# Autodesk Inventor assembly: 0005-00-02 X axis
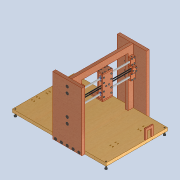
[picture p0: Inventor's stored thumbnail of the model, 180x180]
Saved by Autodesk Inventor 2020 (Build 240168000, 168)
## iProperties
Created: 2020-12-18
Part Number: 0005-00-02 X axis
Document SubType Name: Assembly
Designer: Iulian Bors
Mass: 17144.8 g
Surface Area: 27601.7 cm^2
Volume: 16303.9 cm^3
Density: 1.05157 g/cm^3
Author: Iulian Bors
## Documents named in this file (22)
- Z:\I.A.B\Proiecte\0005 I.A.B 3d 2.0 Imprimanta aracet\10 Mecanic\0005-00-02 X axis.iam
- Z:\I.A.B\Proiecte\0005 I.A.B 3d 2.0 Imprimanta aracet\10 Mecanic\0005-10-011.ipt
- Z:\I.A.B\Proiecte\0005 I.A.B 3d 2.0 Imprimanta aracet\10 Mecanic\0005-10-012.ipt
- Z:\I.A.B\Proiecte\0005 I.A.B 3d 2.0 Imprimanta aracet\10 Mecanic\0005-10-1009 LM10uu.ipt
- Z:\I.A.B\Proiecte\0005 I.A.B 3d 2.0 Imprimanta aracet\10 Mecanic\Surub M4 saiba piulita.iam
- Z:\I.A.B\Proiecte\0005 I.A.B 3d 2.0 Imprimanta aracet\10 Mecanic\0005-10-027 suport nema Z.ipt
- Z:\I.A.B\Proiecte\0005 I.A.B 3d 2.0 Imprimanta aracet\10 Mecanic\0005-10-1007 Bara rectificata.ipt
- Z:\I.A.B\Proiecte\0005 I.A.B 3d 2.0 Imprimanta aracet\10 Mecanic\0005-10-015 suport tija.ipt
- Z:\I.A.B\Proiecte\0005 I.A.B 3d 2.0 Imprimanta aracet\10 Mecanic\0005-10-1001 NEMA17 - Motor de passo.ipt
- Z:\I.A.B\Proiecte\0005 I.A.B 3d 2.0 Imprimanta aracet\10 Mecanic\0005-10-1010 GT2 Timing Pulley 20 Tooth.ipt
- Z:\I.A.B\Proiecte\0005 I.A.B 3d 2.0 Imprimanta aracet\10 Mecanic\0005-10-1011 16T W6 B3 Without T_Shrinkwrap_1.ipt
- Z:\I.A.B\Proiecte\0005 I.A.B 3d 2.0 Imprimanta aracet\10 Mecanic\0005-10-018 intinzator x.ipt
- Z:\I.A.B\Proiecte\0005 I.A.B 3d 2.0 Imprimanta aracet\10 Mecanic\0005-10-1015 curea x.ipt
- Z:\I.A.B\Proiecte\0005 I.A.B 3d 2.0 Imprimanta aracet\10 Mecanic\0005-10-023 Suport motor x.ipt
- C:\Users\40743\Documents\Inventor\Content Center Files\R2020\en-US\ISO 7050 - C-Z(2)\ISO 7050 - ST 3.5 x 22 - C - Z.ipt
- Z:\I.A.B\Proiecte\0005 I.A.B 3d 2.0 Imprimanta aracet\10 Mecanic\0005-10-01 Cadru.iam
- Z:\I.A.B\Proiecte\0005 I.A.B 3d 2.0 Imprimanta aracet\10 Mecanic\Surub M4 saiba piulita 50mm.iam
- Z:\I.A.B\Proiecte\0005 I.A.B 3d 2.0 Imprimanta aracet\10 Mecanic\0005-10-1030 DIN 933 - M4  x 20.ipt
- Z:\I.A.B\Proiecte\0005 I.A.B 3d 2.0 Imprimanta aracet\10 Mecanic\Surub M4 saiba piulita 60mm.iam
- Z:\I.A.B\Proiecte\0005 I.A.B 3d 2.0 Imprimanta aracet\10 Mecanic\0005-10-1032.ipt
- Z:\I.A.B\Proiecte\0005 I.A.B 3d 2.0 Imprimanta aracet\10 Mecanic\0005-10-1020 ISO 7089 - 3 - 140 HV(1).ipt
- Z:\I.A.B\Proiecte\0005 I.A.B 3d 2.0 Imprimanta aracet\10 Mecanic\0005-10-1033 DIN 914 - M5 x 10.ipt
## Components (82 placed, 21 different names)
1. 0005-10-011.ipt:20 — Flush:69, Flush:70, Mate:151, Insert:33, Insert:34
2. 0005-10-011.ipt:24 — Mate:142, Flush:71, Flush:72, Insert:35, Insert:36
3. 0005-10-012.ipt:25 — Flush:22, Flush:25, Flush:26, Mate:40, Mate:56, Mate:57, Mate:71, Mate:72, Flush:44, Mate:142, Mate:151
4. 0005-10-1009 LM10uu.ipt:28 — Flush:22, Mate:49, Mate:56, Mate:57
5. 0005-10-012.ipt:29 — Flush:25, Flush:34, Flush:26, Mate:40, Insert:18, Insert:19, Flush:69, Flush:70, Flush:71, Flush:72, Insert:21, Insert:22, Insert:24, Insert:25, Insert:27, Insert:28, Insert:30, Insert:40
6. 0005-10-1009 LM10uu.ipt:37 — Mate:49, Flush:34, Flush:45, Mate:172
7. 0005-10-1009 LM10uu.ipt:53 — Mate:71, Mate:72, Flush:44, Mate:73
8. 0005-10-1009 LM10uu.ipt:54 — Flush:45, Mate:73, Mate:164
9. Surub M4 saiba piulita.iam:65 [sub-assembly] — Insert:18
10. Surub M4 saiba piulita.iam:67 [sub-assembly] — Insert:19
11. Surub M4 saiba piulita:7 [sub-assembly] — Insert:21
12. Surub M4 saiba piulita:8 [sub-assembly] — Insert:22
13. Surub M4 saiba piulita:10 [sub-assembly] — Insert:24
14. Surub M4 saiba piulita:11 [sub-assembly] — Insert:27
15. Surub M4 saiba piulita:12 [sub-assembly] — Insert:25
16. Surub M4 saiba piulita:15 [sub-assembly] — Insert:28
17. Surub M4 saiba piulita:17 [sub-assembly] — Insert:30
18. 0005-10-1007 Bara rectificata:1 — Mate:172, Mate:173, Flush:75, Mate:176, Flush:77
19. 0005-10-015 suport tija:1 — Mate:165, Mate:166, Mate:167, Mate:171, Flush:74, Flush:76, Insert:43, Insert:51
20. 0005-10-1001 NEMA17 - Motor de passo:1 — Insert:38, Angle:1
21. 0005-10-1010 GT2 Timing Pulley 20 Tooth:1
22. 0005-10-1011 16T W6 B3 Without T_Shrinkwrap_1:1 — Insert:39
23. 0005-10-018 intinzator x:1 — Mate:168, Mate:169, Mate:170, Insert:39, Insert:46, Insert:47, Insert:48
24. 0005-10-1015 curea x:1 — Angle:2
25. 0005-10-023 Suport motor x:1 — Insert:37, Mate:175, Insert:38, Insert:45, Insert:50
26. 0005-10-1007 Bara rectificata:2 — Mate:164, Mate:171, Flush:74, Mate:177, Flush:78
27. 0005-10-01 Cadru:1 [sub-assembly] — Mate:165, Mate:166, Mate:167, Mate:168, Mate:169, Mate:170, Mate:174, Insert:37, Mate:175, Mate:178, Mate:179, Angle:2, Angle:3
28. 0005-10-015 suport tija:2 — Mate:173, Flush:75, Mate:174, Flush:76, Insert:44, Insert:52
29. Surub M4 saiba piulita:18 [sub-assembly] — Insert:40
30. 0005-10-015 suport tija:3 — Mate:176, Flush:77, Mate:179, Insert:41, Insert:54
31. 0005-10-015 suport tija:4 — Mate:177, Flush:78, Mate:178, Insert:42, Insert:53
32. DIN 933 - replaced by DIN EN 24017 M4  x 20:1 — Insert:46
33. Surub M4 saiba piulita 60mm:1 [sub-assembly] — Insert:48
34. Surub M4 saiba piulita 60mm:2 [sub-assembly] — Insert:47
35. DIN 914 M5 x 10:1 — Insert:51
36. DIN 914 M5 x 10:2 — Insert:52
37. DIN 914 M5 x 10:3 — Insert:54
38. DIN 914 M5 x 10:4 — Insert:53
39. ISO 7050 - C-Z ST 3.5 x 22 - C - Z:2 — Insert:34
40. ISO 7050 - C-Z ST 3.5 x 22 - C - Z:5
41. ISO 7050 - C-Z ST 3.5 x 22 - C - Z:6
42. ISO 7050 - C-Z ST 3.5 x 22 - C - Z:7
43. ISO 7050 - C-Z ST 3.5 x 22 - C - Z:1 — Insert:33
44. ISO 7050 - C-Z ST 3.5 x 22 - C - Z:8
45. ISO 7050 - C-Z ST 3.5 x 22 - C - Z:9
46. ISO 7050 - C-Z ST 3.5 x 22 - C - Z:10
47. ISO 7050 - C-Z ST 3.5 x 22 - C - Z:3 — Insert:36
48. ISO 7050 - C-Z ST 3.5 x 22 - C - Z:11
49. ISO 7050 - C-Z ST 3.5 x 22 - C - Z:12
50. ISO 7050 - C-Z ST 3.5 x 22 - C - Z:13
51. ISO 7050 - C-Z ST 3.5 x 22 - C - Z:4 — Insert:35
52. ISO 7050 - C-Z ST 3.5 x 22 - C - Z:14
53. ISO 7050 - C-Z ST 3.5 x 22 - C - Z:15
54. ISO 7050 - C-Z ST 3.5 x 22 - C - Z:16
55. Surub M4 saiba piulita 50mm:1 [sub-assembly] — Insert:41
56. Surub M4 saiba piulita 50mm:3 [sub-assembly]
57. Surub M4 saiba piulita 50mm:4 [sub-assembly]
58. Surub M4 saiba piulita 50mm:5 [sub-assembly]
59. Surub M4 saiba piulita 50mm:2 [sub-assembly] — Insert:42
60. Surub M4 saiba piulita 50mm:7 [sub-assembly]
61. Surub M4 saiba piulita 50mm:8 [sub-assembly]
62. Surub M4 saiba piulita 50mm:9 [sub-assembly]
63. Surub M4 saiba piulita 50mm:6 [sub-assembly] — Insert:43
64. Surub M4 saiba piulita 50mm:11 [sub-assembly]
65. Surub M4 saiba piulita 50mm:12 [sub-assembly]
66. Surub M4 saiba piulita 50mm:13 [sub-assembly]
67. Surub M4 saiba piulita 50mm:10 [sub-assembly] — Insert:44
68. Surub M4 saiba piulita 50mm:14 [sub-assembly]
69. Surub M4 saiba piulita 50mm:15 [sub-assembly]
70. Surub M4 saiba piulita 50mm:16 [sub-assembly]
71. Surub M4 saiba piulita:19 [sub-assembly] — Insert:45
72. Surub M4 saiba piulita:20 [sub-assembly]
73. Surub M4 saiba piulita:21 [sub-assembly] — Angle:3
74. Surub M4 saiba piulita:22 [sub-assembly]
75. DIN 7984 M3 x 16:1 — Insert:49
76. ISO 7089 3:1 — Insert:49, Insert:50
77. DIN 7984 M3 x 16:2
78. ISO 7089 3:2
79. DIN 7984 M3 x 16:3
80. ISO 7089 3:3
81. DIN 7984 M3 x 16:4
82. ISO 7089 3:4
## Component patterns: (4 elements, first: ISO 7050 - C-Z ST 3.5 x 22 - C - Z:2), (4 elements, first: ISO 7050 - C-Z ST 3.5 x 22 - C - Z:1), (4 elements, first: ISO 7050 - C-Z ST 3.5 x 22 - C - Z:3), (4 elements, first: ISO 7050 - C-Z ST 3.5 x 22 - C - Z:4), (4 elements, first: Surub M4 saiba piulita 50mm:1), (4 elements, first: Surub M4 saiba piulita 50mm:2), (4 elements, first: Surub M4 saiba piulita 50mm:6), (4 elements, first: Surub M4 saiba piulita 50mm:10), (4 elements, first: Surub M4 saiba piulita:19), (4 elements, first: DIN 7984 M3 x 16:1 + ISO 7089 3:1)
## Relationships (79: Insert 31, Mate 29, Flush 16, Angle 3)
- Flush:22: 0005-10-012.ipt:25 ↔ 0005-10-1009 LM10uu.ipt:28
- Flush:25: 0005-10-012.ipt:25 ↔ 0005-10-012.ipt:29
- Flush:34: 0005-10-012.ipt:29 ↔ 0005-10-1009 LM10uu.ipt:37
- Flush:26: 0005-10-012.ipt:25 ↔ 0005-10-012.ipt:29
- Mate:40 (19 mm): 0005-10-012.ipt:25 ↔ 0005-10-012.ipt:29
- Mate:49: 0005-10-1009 LM10uu.ipt:28 ↔ 0005-10-1009 LM10uu.ipt:37
- Mate:56 (9.5 mm): 0005-10-012.ipt:25 ↔ 0005-10-1009 LM10uu.ipt:28
- Mate:57 (-30 mm): 0005-10-012.ipt:25 ↔ 0005-10-1009 LM10uu.ipt:28
- Mate:71: 0005-10-012.ipt:25 ↔ 0005-10-1009 LM10uu.ipt:53
- Mate:72 (9.5 mm): 0005-10-012.ipt:25 ↔ 0005-10-1009 LM10uu.ipt:53
- Flush:44 (30 mm): 0005-10-012.ipt:25 ↔ 0005-10-1009 LM10uu.ipt:53
- Flush:45: 0005-10-1009 LM10uu.ipt:37 ↔ 0005-10-1009 LM10uu.ipt:54
- Mate:73: 0005-10-1009 LM10uu.ipt:53 ↔ 0005-10-1009 LM10uu.ipt:54
- Insert:18: 0005-10-012.ipt:29 ↔ Surub M4 saiba piulita.iam:65
- Insert:19: 0005-10-012.ipt:29 ↔ Surub M4 saiba piulita.iam:67
- Flush:69: 0005-10-011.ipt:20 ↔ 0005-10-012.ipt:29
- Flush:70: 0005-10-011.ipt:20 ↔ 0005-10-012.ipt:29
- Mate:142: 0005-10-011.ipt:24 ↔ 0005-10-012.ipt:25
- Flush:71: 0005-10-011.ipt:24 ↔ 0005-10-012.ipt:29
- Flush:72: 0005-10-011.ipt:24 ↔ 0005-10-012.ipt:29
- Mate:151: 0005-10-011.ipt:20 ↔ 0005-10-012.ipt:25
- Insert:21: 0005-10-012.ipt:29 ↔ Surub M4 saiba piulita:7
- Insert:22: 0005-10-012.ipt:29 ↔ Surub M4 saiba piulita:8
- Insert:24: 0005-10-012.ipt:29 ↔ Surub M4 saiba piulita:10
- Insert:25: 0005-10-012.ipt:29 ↔ Surub M4 saiba piulita:12
- Insert:27: 0005-10-012.ipt:29 ↔ Surub M4 saiba piulita:11
- Insert:28: 0005-10-012.ipt:29 ↔ Surub M4 saiba piulita:15
- Insert:30: 0005-10-012.ipt:29 ↔ Surub M4 saiba piulita:17
- [Flush]: 0005-10-1010 GT2 Timing Pulley 20 Tooth:1 ↔ 0005-10-1011 16T W6 B3 Without T_Shrinkwrap_1:1
- [Mate]: 0005-10-1010 GT2 Timing Pulley 20 Tooth:1 ↔ 0005-10-1011 16T W6 B3 Without T_Shrinkwrap_1:1
- [Mate]: 0005-10-1010 GT2 Timing Pulley 20 Tooth:1 ↔ 0005-10-1015 curea x:1
- [Mate]: 0005-10-1010 GT2 Timing Pulley 20 Tooth:1 ↔ 0005-10-1015 curea x:1
- [Mate]: 0005-10-1001 NEMA17 - Motor de passo:1 ↔ 0005-10-1010 GT2 Timing Pulley 20 Tooth:1
- Insert:33: 0005-10-011.ipt:20 ↔ ISO 7050 - C-Z ST 3.5 x 22 - C - Z:1
- Insert:34: 0005-10-011.ipt:20 ↔ ISO 7050 - C-Z ST 3.5 x 22 - C - Z:2
- Insert:35: 0005-10-011.ipt:24 ↔ ISO 7050 - C-Z ST 3.5 x 22 - C - Z:4
- Insert:36: 0005-10-011.ipt:24 ↔ ISO 7050 - C-Z ST 3.5 x 22 - C - Z:3
- Mate:164: 0005-10-1009 LM10uu.ipt:54 ↔ 0005-10-1007 Bara rectificata:2
- Mate:165: 0005-10-015 suport tija:1 ↔ 0005-10-01 Cadru:1
- Mate:166: 0005-10-015 suport tija:1 ↔ 0005-10-01 Cadru:1
- Mate:167: 0005-10-015 suport tija:1 ↔ 0005-10-01 Cadru:1
- Mate:168: 0005-10-018 intinzator x:1 ↔ 0005-10-01 Cadru:1
- Mate:169: 0005-10-018 intinzator x:1 ↔ 0005-10-01 Cadru:1
- Mate:170: 0005-10-018 intinzator x:1 ↔ 0005-10-01 Cadru:1
- Mate:171: 0005-10-015 suport tija:1 ↔ 0005-10-1007 Bara rectificata:2
- Flush:74: 0005-10-015 suport tija:1 ↔ 0005-10-1007 Bara rectificata:2
- Mate:172: 0005-10-1009 LM10uu.ipt:37 ↔ 0005-10-1007 Bara rectificata:1
- Mate:173: 0005-10-1007 Bara rectificata:1 ↔ 0005-10-015 suport tija:2
- Flush:75: 0005-10-1007 Bara rectificata:1 ↔ 0005-10-015 suport tija:2
- Mate:174: 0005-10-01 Cadru:1 ↔ 0005-10-015 suport tija:2
- Flush:76: 0005-10-015 suport tija:1 ↔ 0005-10-015 suport tija:2
- Insert:37: 0005-10-023 Suport motor x:1 ↔ 0005-10-01 Cadru:1
- Mate:175: 0005-10-023 Suport motor x:1 ↔ 0005-10-01 Cadru:1
- Insert:38: 0005-10-1001 NEMA17 - Motor de passo:1 ↔ 0005-10-023 Suport motor x:1
- Angle:1 (0 deg): 0005-10-1001 NEMA17 - Motor de passo:1
- Insert:39 (1 mm): 0005-10-1011 16T W6 B3 Without T_Shrinkwrap_1:1 ↔ 0005-10-018 intinzator x:1
- Insert:40: 0005-10-012.ipt:29 ↔ Surub M4 saiba piulita:18
- Mate:176: 0005-10-1007 Bara rectificata:1 ↔ 0005-10-015 suport tija:3
- Flush:77: 0005-10-1007 Bara rectificata:1 ↔ 0005-10-015 suport tija:3
- Mate:177: 0005-10-1007 Bara rectificata:2 ↔ 0005-10-015 suport tija:4
- Flush:78: 0005-10-1007 Bara rectificata:2 ↔ 0005-10-015 suport tija:4
- Mate:178: 0005-10-01 Cadru:1 ↔ 0005-10-015 suport tija:4
- Mate:179: 0005-10-01 Cadru:1 ↔ 0005-10-015 suport tija:3
- Insert:41: 0005-10-015 suport tija:3 ↔ Surub M4 saiba piulita 50mm:1
- Insert:42: 0005-10-015 suport tija:4 ↔ Surub M4 saiba piulita 50mm:2
- Insert:43: 0005-10-015 suport tija:1 ↔ Surub M4 saiba piulita 50mm:6
- Insert:44: 0005-10-015 suport tija:2 ↔ Surub M4 saiba piulita 50mm:10
- Angle:2 (0 deg): 0005-10-1015 curea x:1 ↔ 0005-10-01 Cadru:1
- Insert:45: 0005-10-023 Suport motor x:1 ↔ Surub M4 saiba piulita:19
- Insert:46: 0005-10-018 intinzator x:1 ↔ DIN 933 - replaced by DIN EN 24017 M4  x 20:1
- Insert:47: 0005-10-018 intinzator x:1 ↔ Surub M4 saiba piulita 60mm:2
- Insert:48: 0005-10-018 intinzator x:1 ↔ Surub M4 saiba piulita 60mm:1
- Insert:49: DIN 7984 M3 x 16:1 ↔ ISO 7089 3:1
- Insert:50: 0005-10-023 Suport motor x:1 ↔ ISO 7089 3:1
- Angle:3 (0 deg): 0005-10-01 Cadru:1 ↔ Surub M4 saiba piulita:21
- Insert:51: 0005-10-015 suport tija:1 ↔ DIN 914 M5 x 10:1
- Insert:52: 0005-10-015 suport tija:2 ↔ DIN 914 M5 x 10:2
- Insert:53: 0005-10-015 suport tija:4 ↔ DIN 914 M5 x 10:4
- Insert:54: 0005-10-015 suport tija:3 ↔ DIN 914 M5 x 10:3
